# Autodesk Inventor assembly: drive
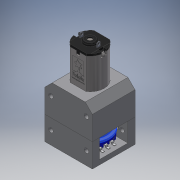
[picture p0: Inventor's stored thumbnail of the model, 180x180]
Saved by Autodesk Inventor 2017 (Build 210142000, 142)
## iProperties
Created: 2018-09-04
Part Number: drive
Document SubType Name: Assembly
Designer: jakub.tomczynski
Author: jakub.tomczynski
## Documents named in this file (8)
- C:\InventorVault-Lider\LiderWorkspace\LiderHand\underactuated finger\drive.iam
- C:\InventorVault-Lider\LiderWorkspace\LiderHand\underactuated finger\drive L.ipt
- C:\InventorVault-Lider\LiderWorkspace\LiderHand\underactuated finger\drive R.ipt
- C:\InventorVault-Lider\LiderWorkspace\LiderHand\underactuated finger\spool.ipt
- C:\InventorVault-Lider\LiderWorkspace\LiderHand\parts\bearing_2x5x1,5.ipt
- C:\InventorVault-Lider\LiderWorkspace\LiderHand\parts\alps_RDC503013A.ipt
- C:\InventorVault-Lider\LiderWorkspace\LiderHand\underactuated finger\drive shaft.ipt
- C:\InventorVault-Lider\LiderWorkspace\LiderHand\parts\micro-metal-gearmotor underactuated drive.ipt
## Components (7 placed, 7 different names)
1. drive L:1 — Flush:1, Flush:2, Flush:3, Mate:1, Mate:2, Mate:3, Mate:9, Mate:10, Mate:11, Mate:12, Mate:13, Flush:4
2. drive R:1 — Mate:1, Mate:15, Flush:4, Mate:16, Mate:17
3. spool:1 — Mate:6, Mate:7
4. bearing_2x5x1,5:1 — Mate:2, Mate:3, Mate:4, Mate:5
5. alps_RDC503013A:1 — Mate:8, Mate:9, Mate:10, Mate:11, Mate:12, Mate:13
6. drive shaft:1 — Mate:4, Mate:5, Mate:6, Mate:7, Mate:8, Mate:14
7. micro-metal-gearmotor underactuated drive:1 — Mate:14, Mate:15, Mate:16, Mate:17
## Relationships (21: Mate 17, Flush 4)
- Flush:1: drive L:1
- Flush:2: drive L:1
- Flush:3: drive L:1
- Mate:1: drive L:1 ↔ drive R:1
- Mate:2: drive L:1 ↔ bearing_2x5x1,5:1
- Mate:3: drive L:1 ↔ bearing_2x5x1,5:1
- Mate:4: bearing_2x5x1,5:1 ↔ drive shaft:1
- Mate:5: bearing_2x5x1,5:1 ↔ drive shaft:1
- Mate:6: spool:1 ↔ drive shaft:1
- Mate:7: spool:1 ↔ drive shaft:1
- Mate:8: alps_RDC503013A:1 ↔ drive shaft:1
- Mate:9: drive L:1 ↔ alps_RDC503013A:1
- Mate:10: drive L:1 ↔ alps_RDC503013A:1
- Mate:11: drive L:1 ↔ alps_RDC503013A:1
- Mate:12: drive L:1 ↔ alps_RDC503013A:1
- Mate:13: drive L:1 ↔ alps_RDC503013A:1
- Mate:14: drive shaft:1 ↔ micro-metal-gearmotor underactuated drive:1
- Mate:15: drive R:1 ↔ micro-metal-gearmotor underactuated drive:1
- Flush:4: drive L:1 ↔ drive R:1
- Mate:16: drive R:1 ↔ micro-metal-gearmotor underactuated drive:1
- Mate:17: drive R:1 ↔ micro-metal-gearmotor underactuated drive:1
